# Autodesk Inventor assembly: Intake
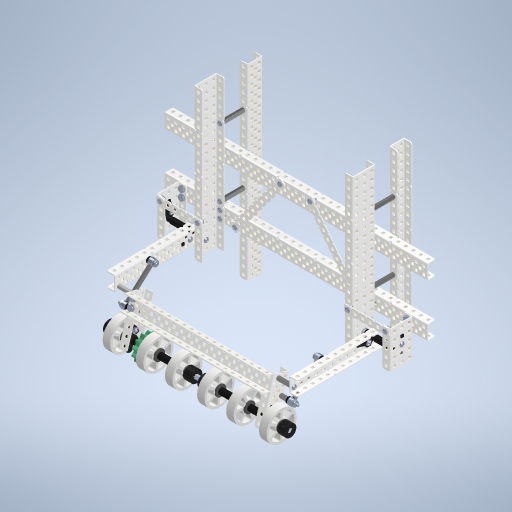
[picture p0: Inventor's stored thumbnail of the model, 512x512]
Saved by Autodesk Inventor 2023 (Build 270158000, 158)
## iProperties
Created: 2022-09-02
Part Number: Intake
Document SubType Name: Assembly
Designer: alex
Author: alex
## Documents named in this file (26)
- C:\Users\alex\Documents\GitHub\4067X_spin_up_cad\Mechanism\Intake.iam
- C:\Users\alex\Documents\GitHub\4067X_spin_up_cad\Library\Structure\Standoff\Standoff 1.00.ipt
- C:\Users\alex\Documents\GitHub\4067X_spin_up_cad\Library\Structure\Standoff.ipt
- C:\Users\alex\Documents\GitHub\4067X_spin_up_cad\Library\Structure\Hardware\Screw Steel - Star\SScrew Star Smooth .290.ipt
- C:\Users\alex\Documents\GitHub\4067X_spin_up_cad\Library\Structure\Hardware\Screw Steel - Star.ipt
- C:\Users\alex\Documents\GitHub\4067X_spin_up_cad\Library\Structure\Standoff\Standoff .50.ipt
- C:\Users\alex\Documents\GitHub\4067X_spin_up_cad\Library\Motion\Spacers\Spacer Nylon .375 OD.ipt
- C:\Users\alex\Documents\GitHub\4067X_spin_up_cad\Library\Structure\Hardware\Nut Keps.ipt
- C:\Users\alex\Documents\GitHub\4067X_spin_up_cad\Library\Motion\1-Post Bearing Flat Hex Retainer.ipt
- C:\Users\alex\Documents\GitHub\4067X_spin_up_cad\Library\Structure\Hardware\Screw Steel - Star\SScrew Star Smooth .375.ipt
- C:\Users\alex\Documents\GitHub\4067X_spin_up_cad\Library\Structure\Hardware\Nut Nylock.ipt
- C:\Users\alex\Documents\GitHub\4067X_spin_up_cad\Library\Structure\C-Channels\Aluminum 1x3x1\Alu C 1x3x1x20.ipt
- C:\Users\alex\Documents\GitHub\4067X_spin_up_cad\Library\Structure\C-Channels\Aluminum 1x3x1\Alu C 1x3x1x5.ipt
- C:\Users\alex\Documents\GitHub\4067X_spin_up_cad\Library\Structure\C-Channels\Aluminum 1x2x1\Alu C 1x2x1x35.ipt
- C:\Users\alex\Documents\GitHub\4067X_spin_up_cad\Library\Structure\Hardware\Screw Steel - Star\SScrew Star Smooth 2.500.ipt
- C:\Users\alex\Documents\GitHub\4067X_spin_up_cad\Library\Motion\Spacers\Spacer Nylon .375 OD\NSpacer .375 OD x .375.ipt
- C:\Users\alex\Documents\GitHub\4067X_spin_up_cad\Library\Motion\Spacers\Spacer Nylon .375 OD\NSpacer .375 OD x .500.ipt
- C:\Users\alex\Documents\GitHub\4067X_spin_up_cad\Library\Structure\C-Channels\Aluminum 1x2x1\Alu C 1x2x1x25.ipt
- C:\Users\alex\Documents\GitHub\4067X_spin_up_cad\Library\Structure\Hardware\Screw Steel - Star\SScrew Star Smooth .750.ipt
- C:\Users\alex\Documents\GitHub\4067X_spin_up_cad\Mechanism\FloatingIntake.iam
- C:\Users\alex\Documents\GitHub\4067X_spin_up_cad\Library\Motion\Spacers\Spacer Nylon .375 OD\NSpacer .375 OD x .250.ipt
- C:\Users\alex\Documents\GitHub\4067X_spin_up_cad\Library\Motion\Spacers\Washer Teflon\TWasher .375 OD x .06250.ipt
- C:\Users\alex\Documents\GitHub\4067X_spin_up_cad\Library\Motion\Spacers\Washer Teflon.ipt
- C:\Users\alex\Documents\GitHub\4067X_spin_up_cad\Library\Motion\Spacers\Washer Teflon\TWasher .375 OD x .04000.ipt
- C:\Users\alex\Documents\GitHub\4067X_spin_up_cad\Library\Structure\Plates\Aluminum\VEX Plates\Alu Plate VEX 1x11.ipt
- C:\Users\alex\Documents\GitHub\4067X_spin_up_cad\Library\Structure\Plates\Aluminum\VEX Plates\Alu Plate VEX 1x6.ipt
## Components (83 placed, 21 different names)
1. Alu C 1x3x1x5:1 — Insert:107, Insert:108, Insert:120, Mate:15, Insert:145, Insert:230, Insert:244, Insert:245, Insert:298
2. Alu C 1x2x1x35:1 — Insert:107, Insert:108, Insert:150, Insert:151, Insert:218, Insert:219, Insert:236, Insert:237, Insert:252, Insert:253, Insert:277, Insert:278, Insert:285, Insert:286, Insert:304, Insert:305, Insert:309, Insert:313, Insert:314, Insert:317
3. Standoff 1.00:16 — Insert:110, Insert:287
4. Standoff .50:17 — Insert:110, Insert:125
5. Standoff 1.00:18 — Insert:288
6. Standoff .50:19 — Insert:124
7. 1-Post Bearing Flat Hex Retainer:2 — Insert:120, Mate:15, Insert:146
8. NSpacer .375 OD x .500:4 — Insert:122, Insert:294
9. NSpacer .375 OD x .500:5 — Insert:122, Insert:123
10. NSpacer .375 OD x .375:6 — Insert:123
11. Alu C 1x2x1x25:1 — Insert:124, Insert:125, Insert:239, Insert:240
12. Alu C 1x3x1x20:2 — Insert:252, Insert:253, Mate:35, Insert:254, Insert:255, Insert:260, Insert:263, Insert:267, Insert:268, Insert:275, Insert:276, Insert:280, Insert:283, Insert:284
13. Standoff 1.00:20 — Insert:260
14. Standoff .50:21 — Insert:133
15. Standoff 1.00:22
16. Standoff .50:23 — Insert:132
17. Alu C 1x2x1x25:2 — Insert:132, Insert:133, Insert:227, Insert:243
18. NSpacer .375 OD x .500:8 — Insert:259
19. NSpacer .375 OD x .500:9
20. NSpacer .375 OD x .375:10
21. SScrew Star Smooth .375:34 — Insert:145
22. Nut Nylock:3 — Insert:146
23. Alu C 1x3x1x5:2 — Insert:150, Insert:151, Insert:217, Insert:220, Insert:221, Insert:279
24. 1-Post Bearing Flat Hex Retainer:4
25. SScrew Star Smooth .375:35
26. Nut Nylock:4
27. Nut Keps:12 — Insert:217
28. SScrew Star Smooth .290:52 — Insert:218
29. SScrew Star Smooth .290:53 — Insert:219
30. Nut Keps:13 — Insert:220
31. Nut Keps:14 — Insert:221
32. SScrew Star Smooth .750:57 — Insert:227
33. Nut Keps:17 — Insert:230
34. SScrew Star Smooth .290:62 — Insert:236
35. SScrew Star Smooth .290:63 — Insert:237
36. SScrew Star Smooth .750:65 — Insert:239
37. SScrew Star Smooth .750:66 — Insert:240
38. SScrew Star Smooth .750:69 — Insert:243
39. Nut Keps:21 — Insert:244
40. Nut Keps:22 — Insert:245
41. FloatingIntake:1 [sub-assembly] — Mate:35, Mate:36, Insert:259, Mate:37, Insert:294
42. SScrew Star Smooth 2.500:75 — Insert:254, Mate:36
43. Nut Keps:23 — Insert:255, Insert:256
44. NSpacer .375 OD x .250:11 — Insert:256, Insert:257
45. TWasher .375 OD x .06250:1 — Insert:257, Insert:258
46. TWasher .375 OD x .04000:2 — Insert:258
47. SScrew Star Smooth .290:78 — Insert:263
48. Alu C 1x2x1x35:2 — Insert:267, Insert:268, Insert:308, Insert:312, Insert:315, Insert:316
49. SScrew Star Smooth .290:82 — Insert:275
50. SScrew Star Smooth .290:83 — Insert:276
51. Nut Keps:28 — Insert:277
52. Nut Keps:29 — Insert:278
53. Alu Plate VEX 1x6:1 — Insert:279, Insert:280, Insert:281, Insert:282
54. SScrew Star Smooth .290:84 — Insert:281
55. SScrew Star Smooth .290:85 — Insert:282
56. Nut Keps:30 — Insert:283
57. SScrew Star Smooth .290:86 — Insert:284
58. Alu C 1x3x1x20:3 — Insert:285, Insert:286, Insert:287, Insert:288, Mate:37, Insert:289, Insert:293, Insert:297, Insert:299, Insert:300, Insert:301, Insert:302, Insert:303
59. SScrew Star Smooth 2.500:87 — Insert:289
60. Nut Keps:31 — Insert:293
61. NSpacer .375 OD x .250:12
62. TWasher .375 OD x .06250:3
63. TWasher .375 OD x .04000:4
64. Alu Plate VEX 1x6:2 — Insert:297, Insert:298
65. SScrew Star Smooth .290:88
66. SScrew Star Smooth .290:89
67. Nut Keps:32 — Insert:299
68. SScrew Star Smooth .290:90 — Insert:300
69. SScrew Star Smooth .290:91 — Insert:301
70. SScrew Star Smooth .290:92 — Insert:302
71. SScrew Star Smooth .290:93 — Insert:303
72. Nut Keps:33 — Insert:304
73. Nut Keps:34 — Insert:305
74. Alu Plate VEX 1x11:2 — Insert:308, Insert:309
75. SScrew Star Smooth .290:94
76. SScrew Star Smooth .290:95
77. Alu Plate VEX 1x11:3 — Insert:312, Insert:313
78. SScrew Star Smooth .290:96
79. SScrew Star Smooth .290:97
80. Nut Keps:35 — Insert:314
81. Nut Keps:36 — Insert:315
82. Nut Keps:37 — Insert:316
83. Nut Keps:38 — Insert:317
## Relationships (96: Insert 91, Mate 5)
- Insert:107: Alu C 1x3x1x5:1 ↔ Alu C 1x2x1x35:1
- Insert:108: Alu C 1x3x1x5:1 ↔ Alu C 1x2x1x35:1
- Insert:110: Standoff 1.00:16 ↔ Standoff .50:17
- [Insert]: Standoff 1.00:18 ↔ Standoff .50:19
- Insert:120: Alu C 1x3x1x5:1 ↔ 1-Post Bearing Flat Hex Retainer:2
- Mate:15: Alu C 1x3x1x5:1 ↔ 1-Post Bearing Flat Hex Retainer:2
- Insert:122: NSpacer .375 OD x .500:4 ↔ NSpacer .375 OD x .500:5
- Insert:123: NSpacer .375 OD x .500:5 ↔ NSpacer .375 OD x .375:6
- Insert:124: Standoff .50:19 ↔ Alu C 1x2x1x25:1
- Insert:125: Standoff .50:17 ↔ Alu C 1x2x1x25:1
- [Insert]: Standoff 1.00:20 ↔ Standoff .50:21
- [Insert]: Standoff 1.00:22 ↔ Standoff .50:23
- Insert:132: Standoff .50:23 ↔ Alu C 1x2x1x25:2
- Insert:133: Standoff .50:21 ↔ Alu C 1x2x1x25:2
- [Insert]: NSpacer .375 OD x .500:8 ↔ NSpacer .375 OD x .500:9
- [Insert]: NSpacer .375 OD x .500:9 ↔ NSpacer .375 OD x .375:10
- Insert:145: Alu C 1x3x1x5:1 ↔ SScrew Star Smooth .375:34
- Insert:146: 1-Post Bearing Flat Hex Retainer:2 ↔ Nut Nylock:3
- [Insert]: Alu C 1x3x1x5:2 ↔ 1-Post Bearing Flat Hex Retainer:4
- [Mate]: Alu C 1x3x1x5:2 ↔ 1-Post Bearing Flat Hex Retainer:4
- [Insert]: Alu C 1x3x1x5:2 ↔ SScrew Star Smooth .375:35
- [Insert]: 1-Post Bearing Flat Hex Retainer:4 ↔ Nut Nylock:4
- Insert:150: Alu C 1x2x1x35:1 ↔ Alu C 1x3x1x5:2
- Insert:151: Alu C 1x2x1x35:1 ↔ Alu C 1x3x1x5:2
- Insert:217: Alu C 1x3x1x5:2 ↔ Nut Keps:12
- Insert:218: Alu C 1x2x1x35:1 ↔ SScrew Star Smooth .290:52
- Insert:219: Alu C 1x2x1x35:1 ↔ SScrew Star Smooth .290:53
- Insert:220: Alu C 1x3x1x5:2 ↔ Nut Keps:13
- Insert:221: Alu C 1x3x1x5:2 ↔ Nut Keps:14
- Insert:227: Alu C 1x2x1x25:2 ↔ SScrew Star Smooth .750:57
- Insert:230: Alu C 1x3x1x5:1 ↔ Nut Keps:17
- Insert:236: Alu C 1x2x1x35:1 ↔ SScrew Star Smooth .290:62
- Insert:237: Alu C 1x2x1x35:1 ↔ SScrew Star Smooth .290:63
- Insert:239: Alu C 1x2x1x25:1 ↔ SScrew Star Smooth .750:65
- Insert:240: Alu C 1x2x1x25:1 ↔ SScrew Star Smooth .750:66
- Insert:243: Alu C 1x2x1x25:2 ↔ SScrew Star Smooth .750:69
- Insert:244: Alu C 1x3x1x5:1 ↔ Nut Keps:21
- Insert:245: Alu C 1x3x1x5:1 ↔ Nut Keps:22
- Insert:252: Alu C 1x2x1x35:1 ↔ Alu C 1x3x1x20:2
- Insert:253: Alu C 1x2x1x35:1 ↔ Alu C 1x3x1x20:2
- Mate:35 (12.7 mm): Alu C 1x3x1x20:2 ↔ FloatingIntake:1
- Insert:254: Alu C 1x3x1x20:2 ↔ SScrew Star Smooth 2.500:75
- Insert:255: Alu C 1x3x1x20:2 ↔ Nut Keps:23
- Mate:36: FloatingIntake:1 ↔ SScrew Star Smooth 2.500:75
- Insert:256: Nut Keps:23 ↔ NSpacer .375 OD x .250:11
- Insert:257: NSpacer .375 OD x .250:11 ↔ TWasher .375 OD x .06250:1
- Insert:258: TWasher .375 OD x .06250:1 ↔ TWasher .375 OD x .04000:2
- Insert:259: NSpacer .375 OD x .500:8 ↔ FloatingIntake:1
- Insert:260: Alu C 1x3x1x20:2 ↔ Standoff 1.00:20
- Insert:263: Alu C 1x3x1x20:2 ↔ SScrew Star Smooth .290:78
- Insert:267: Alu C 1x3x1x20:2 ↔ Alu C 1x2x1x35:2
- Insert:268: Alu C 1x3x1x20:2 ↔ Alu C 1x2x1x35:2
- Insert:275: Alu C 1x3x1x20:2 ↔ SScrew Star Smooth .290:82
- Insert:276: Alu C 1x3x1x20:2 ↔ SScrew Star Smooth .290:83
- Insert:277: Alu C 1x2x1x35:1 ↔ Nut Keps:28
- Insert:278: Alu C 1x2x1x35:1 ↔ Nut Keps:29
- Insert:279: Alu C 1x3x1x5:2 ↔ Alu Plate VEX 1x6:1
- Insert:280: Alu C 1x3x1x20:2 ↔ Alu Plate VEX 1x6:1
- Insert:281: Alu Plate VEX 1x6:1 ↔ SScrew Star Smooth .290:84
- Insert:282: Alu Plate VEX 1x6:1 ↔ SScrew Star Smooth .290:85
- Insert:283: Alu C 1x3x1x20:2 ↔ Nut Keps:30
- Insert:284: Alu C 1x3x1x20:2 ↔ SScrew Star Smooth .290:86
- Insert:285: Alu C 1x2x1x35:1 ↔ Alu C 1x3x1x20:3
- Insert:286: Alu C 1x2x1x35:1 ↔ Alu C 1x3x1x20:3
- Insert:287: Standoff 1.00:16 ↔ Alu C 1x3x1x20:3
- Insert:288: Standoff 1.00:18 ↔ Alu C 1x3x1x20:3
- Mate:37 (12.7 mm): FloatingIntake:1 ↔ Alu C 1x3x1x20:3
- Insert:289: Alu C 1x3x1x20:3 ↔ SScrew Star Smooth 2.500:87
- [Insert]: Nut Keps:31 ↔ NSpacer .375 OD x .250:12
- [Insert]: NSpacer .375 OD x .250:12 ↔ TWasher .375 OD x .06250:3
- [Insert]: TWasher .375 OD x .06250:3 ↔ TWasher .375 OD x .04000:4
- Insert:293: Alu C 1x3x1x20:3 ↔ Nut Keps:31
- Insert:294: NSpacer .375 OD x .500:4 ↔ FloatingIntake:1
- [Insert]: Alu Plate VEX 1x6:2 ↔ SScrew Star Smooth .290:88
- [Insert]: Alu Plate VEX 1x6:2 ↔ SScrew Star Smooth .290:89
- Insert:297: Alu C 1x3x1x20:3 ↔ Alu Plate VEX 1x6:2
- Insert:298: Alu C 1x3x1x5:1 ↔ Alu Plate VEX 1x6:2
- Insert:299: Alu C 1x3x1x20:3 ↔ Nut Keps:32
- Insert:300: Alu C 1x3x1x20:3 ↔ SScrew Star Smooth .290:90
- Insert:301: Alu C 1x3x1x20:3 ↔ SScrew Star Smooth .290:91
- Insert:302: Alu C 1x3x1x20:3 ↔ SScrew Star Smooth .290:92
- Insert:303: Alu C 1x3x1x20:3 ↔ SScrew Star Smooth .290:93
- Insert:304: Alu C 1x2x1x35:1 ↔ Nut Keps:33
- Insert:305: Alu C 1x2x1x35:1 ↔ Nut Keps:34
- [Insert]: Alu Plate VEX 1x11:2 ↔ SScrew Star Smooth .290:94
- [Insert]: Alu Plate VEX 1x11:2 ↔ SScrew Star Smooth .290:95
- Insert:308: Alu C 1x2x1x35:2 ↔ Alu Plate VEX 1x11:2
- Insert:309: Alu C 1x2x1x35:1 ↔ Alu Plate VEX 1x11:2
- [Insert]: Alu Plate VEX 1x11:3 ↔ SScrew Star Smooth .290:96
- [Insert]: Alu Plate VEX 1x11:3 ↔ SScrew Star Smooth .290:97
- Insert:312: Alu C 1x2x1x35:2 ↔ Alu Plate VEX 1x11:3
- Insert:313: Alu C 1x2x1x35:1 ↔ Alu Plate VEX 1x11:3
- Insert:314: Alu C 1x2x1x35:1 ↔ Nut Keps:35
- Insert:315: Alu C 1x2x1x35:2 ↔ Nut Keps:36
- Insert:316: Alu C 1x2x1x35:2 ↔ Nut Keps:37
- Insert:317: Alu C 1x2x1x35:1 ↔ Nut Keps:38
## Named parameters: d171_d169 = 0 mm, d195_d169 = 0 mm, d197_d195_d169 = 0 mm, d210_d188 = 0 mm, d211_d189 = 0 mm, d215_d185 = 0 mm, d216_d186 = 0 mm, d217_d213 = 0 mm, d218_d214 = 0 mm, d407_d369 = 0 mm, d408_d370 = 0 mm, d409_d371 = 0 mm, d412_d396 = 0 mm, d413_d397 = 0 mm, d423_d386 = 0 mm, d424_d387 = 0 mm, d427_d423_d386 = 0 mm, d428_d424_d387 = 0 mm
